# Autodesk Inventor assembly: Drive Tube Assem
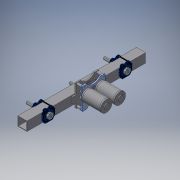
[picture p0: Inventor's stored thumbnail of the model, 180x180]
Saved by Autodesk Inventor 2019 (Build 230136000, 136)
## iProperties
Created: 2018-11-11
Part Number: Drive Tube Assem
Document SubType Name: Assembly
Designer: maste
Author: maste
## Documents named in this file (7)
- D:\Summer Drive Base V1\Summer Drivebase\Drive Tube Assem.iam
- D:\Summer Drive Base V1\Summer Drivebase\2x2 26in.ipt
- D:\Summer Drive Base V1\Summer Drivebase\Bearing Block Assem.iam
- D:\Summer Drive Base V1\Summer Drivebase\1in Spacer.ipt
- D:\Summer Drive Base V1\Summer Drivebase\0.0625in Spacer.ipt
- D:\Summer Drive Base V1\Summer Drivebase\36t_x_9mm_Wide_Double_Flange_Aluminum_Pulley_GT2_3mm_1_2_Hex_Bore_217-5873.ipt
- D:\Summer Drive Base V1\Summer Drivebase\Gearbox.iam
## Components (12 placed, 6 different names)
1. 2x2 26in:1 — Mate:1, Mate:2, Mate:3, Mate:4, Mate:5, Mate:6, Mate:27, Mate:28, Mate:29, Rotation:1
2. Bearing Block Assem:1 [sub-assembly] — Mate:4, Mate:5, Mate:6, Mate:7, Mate:8, Mate:9, Mate:14, Mate:17, Mate:18, Mate:20, Mate:21
3. Bearing Block Assem:2 [sub-assembly] — Mate:1, Mate:2, Mate:3, Mate:10, Mate:11, Mate:12, Mate:24, Mate:25, Mate:26
4. 1in Spacer:1 — Mate:10, Mate:11, Mate:12
5. 1in Spacer:2 — Mate:7, Mate:8, Mate:9, Mate:13, Mate:15
6. 0.0625in Spacer:1 — Mate:13, Mate:14, Mate:15, Mate:16
7. 0.0625in Spacer:2 — Mate:23, Flush:3, Flush:4
8. 36t_x_9mm_Wide_Double_Flange_Aluminum_Pulley_GT2_3mm_1_2_Hex_Bore_217-5873:1 — Mate:22, Flush:1, Flush:2, Mate:23, Flush:3, Flush:4
9. 36t_x_9mm_Wide_Double_Flange_Aluminum_Pulley_GT2_3mm_1_2_Hex_Bore_217-5873:2 — Mate:16, Mate:17, Mate:18, Mate:19
10. 0.0625in Spacer:3 — Mate:19, Mate:20, Mate:21
11. 0.0625in Spacer:4 — Mate:22, Flush:1, Flush:2, Mate:24, Mate:25, Mate:26
12. Gearbox:1 [sub-assembly] — Mate:27, Mate:28, Mate:29, Rotation:1
## Relationships (34: Mate 29, Flush 4, RelateRotation 1)
- Mate:1: 2x2 26in:1 ↔ Bearing Block Assem:2
- Mate:2: 2x2 26in:1 ↔ Bearing Block Assem:2
- Mate:3: 2x2 26in:1 ↔ Bearing Block Assem:2
- Mate:4: 2x2 26in:1 ↔ Bearing Block Assem:1
- Mate:5: 2x2 26in:1 ↔ Bearing Block Assem:1
- Mate:6: 2x2 26in:1 ↔ Bearing Block Assem:1
- Mate:7: Bearing Block Assem:1 ↔ 1in Spacer:2
- Mate:8: Bearing Block Assem:1 ↔ 1in Spacer:2
- Mate:9: Bearing Block Assem:1 ↔ 1in Spacer:2
- Mate:10: Bearing Block Assem:2 ↔ 1in Spacer:1
- Mate:11: Bearing Block Assem:2 ↔ 1in Spacer:1
- Mate:12: Bearing Block Assem:2 ↔ 1in Spacer:1
- Mate:13: 1in Spacer:2 ↔ 0.0625in Spacer:1
- Mate:14: Bearing Block Assem:1 ↔ 0.0625in Spacer:1
- Mate:15: 1in Spacer:2 ↔ 0.0625in Spacer:1
- Mate:16: 0.0625in Spacer:1 ↔ 36t_x_9mm_Wide_Double_Flange_Aluminum_Pulley_GT2_3mm_1_2_Hex_Bore_217-5873:2
- Mate:17: Bearing Block Assem:1 ↔ 36t_x_9mm_Wide_Double_Flange_Aluminum_Pulley_GT2_3mm_1_2_Hex_Bore_217-5873:2
- Mate:18: Bearing Block Assem:1 ↔ 36t_x_9mm_Wide_Double_Flange_Aluminum_Pulley_GT2_3mm_1_2_Hex_Bore_217-5873:2
- Mate:19: 36t_x_9mm_Wide_Double_Flange_Aluminum_Pulley_GT2_3mm_1_2_Hex_Bore_217-5873:2 ↔ 0.0625in Spacer:3
- Mate:20: Bearing Block Assem:1 ↔ 0.0625in Spacer:3
- Mate:21: Bearing Block Assem:1 ↔ 0.0625in Spacer:3
- Mate:22: 36t_x_9mm_Wide_Double_Flange_Aluminum_Pulley_GT2_3mm_1_2_Hex_Bore_217-5873:1 ↔ 0.0625in Spacer:4
- Flush:1: 36t_x_9mm_Wide_Double_Flange_Aluminum_Pulley_GT2_3mm_1_2_Hex_Bore_217-5873:1 ↔ 0.0625in Spacer:4
- Flush:2: 36t_x_9mm_Wide_Double_Flange_Aluminum_Pulley_GT2_3mm_1_2_Hex_Bore_217-5873:1 ↔ 0.0625in Spacer:4
- Mate:23: 0.0625in Spacer:2 ↔ 36t_x_9mm_Wide_Double_Flange_Aluminum_Pulley_GT2_3mm_1_2_Hex_Bore_217-5873:1
- Flush:3: 0.0625in Spacer:2 ↔ 36t_x_9mm_Wide_Double_Flange_Aluminum_Pulley_GT2_3mm_1_2_Hex_Bore_217-5873:1
- Flush:4: 0.0625in Spacer:2 ↔ 36t_x_9mm_Wide_Double_Flange_Aluminum_Pulley_GT2_3mm_1_2_Hex_Bore_217-5873:1
- Mate:24: Bearing Block Assem:2 ↔ 0.0625in Spacer:4
- Mate:25: Bearing Block Assem:2 ↔ 0.0625in Spacer:4
- Mate:26: Bearing Block Assem:2 ↔ 0.0625in Spacer:4
- Mate:27: 2x2 26in:1 ↔ Gearbox:1
- Mate:28: 2x2 26in:1 ↔ Gearbox:1
- Mate:29: 2x2 26in:1 ↔ Gearbox:1
- Rotation:1 [RelateRotation] (1 ul): 2x2 26in:1 ↔ Gearbox:1
